# Autodesk Inventor assembly: BlueCrowsNestFinal-ver1-1111-2021
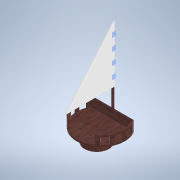
[picture p0: Inventor's stored thumbnail of the model, 180x180]
Saved by Autodesk Inventor 2021 (Build 250183000, 183)
## iProperties
Created: 2021-03-02
Part Number: BlueCrowsNestFinal-ver1-1111-2021
Document SubType Name: Assembly
Designer: CMurray
Author: CMurray
## Documents named in this file (8)
- F:\PHRC CADD 2021\2021 Game Design Challenge\Crow's Nest\Assemblies\BlueCrowsNestFinal-ver1-1111-2021.iam
- F:\PHRC CADD 2021\2021 Game Design Challenge\Crow's Nest\Parts\Nest-ver3-1111-2021.ipt
- F:\PHRC CADD 2021\2021 Game Design Challenge\Crow's Nest\Parts\NestTop-ver2-1111-2021.ipt
- F:\PHRC CADD 2021\2021 Game Design Challenge\Crow's Nest\Parts\NestPost-ver1-1111-2021.ipt
- F:\PHRC CADD 2021\2021 Game Design Challenge\Crow's Nest\Parts\WinchWall-ver1-1111-2021.ipt
- F:\PHRC CADD 2021\2021 Game Design Challenge\Sail\Parts\SailPost-ver3-1111-2021.ipt
- F:\PHRC CADD 2021\2021 Game Design Challenge\Sail\Assemblies\FinalRedSail-ver1-1111-2021.iam
- F:\PHRC CADD 2021\2021 Game Design Challenge\Sail\Assemblies\FinalBlueSail-ver1-1111-2021.iam
## Components (7 placed, 7 different names)
1. Nest-ver3-1111-2021:1 — Mate:1, Flush:1, Mate:2, Mate:3, Mate:4, Angle:1, Mate:5, Angle:2, Mate:6, Angle:3, Mate:7, Angle:4, Mate:8, Angle:5, Flush:2, Mate:9, Mate:10, Mate:14, Mate:15
2. NestTop-ver2-1111-2021:1 — Mate:1, Flush:1, Mate:2, Mate:11, Flush:3, Mate:12
3. NestPost-ver1-1111-2021:1 — Mate:3
4. WinchWall-ver1-1111-2021:1 — Flush:2, Mate:9, Mate:10
5. SailPost-ver3-1111-2021:1 — Mate:11, Flush:3, Mate:12, Mate:13, Flush:4, Flush:5
6. FinalRedSail-ver1-1111-2021:1 [sub-assembly] — Mate:13, Flush:4, Mate:14
7. FinalBlueSail-ver1-1111-2021:1 [sub-assembly] — Mate:15, Flush:5
## Relationships (25: Mate 15, Flush 5, Angle 5)
- Mate:1: Nest-ver3-1111-2021:1 ↔ NestTop-ver2-1111-2021:1
- Flush:1: Nest-ver3-1111-2021:1 ↔ NestTop-ver2-1111-2021:1
- Mate:2: Nest-ver3-1111-2021:1 ↔ NestTop-ver2-1111-2021:1
- Mate:3: Nest-ver3-1111-2021:1 ↔ NestPost-ver1-1111-2021:1
- Mate:4: Nest-ver3-1111-2021:1
- Angle:1 (0 deg): Nest-ver3-1111-2021:1
- Mate:5: Nest-ver3-1111-2021:1
- Angle:2 (0 deg): Nest-ver3-1111-2021:1
- Mate:6: Nest-ver3-1111-2021:1
- Angle:3 (0 deg): Nest-ver3-1111-2021:1
- Mate:7: Nest-ver3-1111-2021:1
- Angle:4 (0 deg): Nest-ver3-1111-2021:1
- Mate:8: Nest-ver3-1111-2021:1
- Angle:5 (0 deg): Nest-ver3-1111-2021:1
- Flush:2: Nest-ver3-1111-2021:1 ↔ WinchWall-ver1-1111-2021:1
- Mate:9: Nest-ver3-1111-2021:1 ↔ WinchWall-ver1-1111-2021:1
- Mate:10 (444.5 mm): Nest-ver3-1111-2021:1 ↔ WinchWall-ver1-1111-2021:1
- Mate:11: NestTop-ver2-1111-2021:1 ↔ SailPost-ver3-1111-2021:1
- Flush:3: NestTop-ver2-1111-2021:1 ↔ SailPost-ver3-1111-2021:1
- Mate:12 (736.6 mm): NestTop-ver2-1111-2021:1 ↔ SailPost-ver3-1111-2021:1
- Mate:13 (-57.15 mm): SailPost-ver3-1111-2021:1 ↔ FinalRedSail-ver1-1111-2021:1
- Flush:4 (-12.7 mm): SailPost-ver3-1111-2021:1 ↔ FinalRedSail-ver1-1111-2021:1
- Mate:14 (1016 mm): Nest-ver3-1111-2021:1 ↔ FinalRedSail-ver1-1111-2021:1
- Mate:15 (1016 mm): Nest-ver3-1111-2021:1 ↔ FinalBlueSail-ver1-1111-2021:1
- Flush:5 (-12.7 mm): SailPost-ver3-1111-2021:1 ↔ FinalBlueSail-ver1-1111-2021:1
